# Autodesk Inventor assembly: cycloid_assy
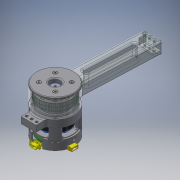
[picture p0: Inventor's stored thumbnail of the model, 180x180]
Saved by Autodesk Inventor 2019.4 (Build 234330000, 330)
## iProperties
Created: 2019-08-28
Part Number: cycloid_assy
Document SubType Name: Assembly
Designer: cdi
Author: cdi
## Documents named in this file (20)
- D:\SynologyDrive\workspace_inventor\2019_06_19.MT4008_actuator\[github_upload]\3d_print_cycloid_actuator_v2\inventor_file\cycloid_assy_v2.iam
- D:\SynologyDrive\workspace_inventor\2019_06_19.MT4008_actuator\[github_upload]\3d_print_cycloid_actuator_v2\inventor_file\bearing_18x12x4.ipt
- D:\SynologyDrive\workspace_inventor\2019_06_19.MT4008_actuator\[github_upload]\3d_print_cycloid_actuator_v2\inventor_file\cycloid_top_bottom_assy.iam
- D:\SynologyDrive\workspace_inventor\2019_06_19.MT4008_actuator\[github_upload]\3d_print_cycloid_actuator_v2\inventor_file\tarot-mt4008-motor-1.snapshot.3\inventor_export\Tarot 4008 Motor Assembly.iam
- D:\SynologyDrive\workspace_inventor\2019_06_19.MT4008_actuator\[github_upload]\3d_print_cycloid_actuator_v2\inventor_file\cycloid_housing.ipt
- D:\SynologyDrive\workspace_inventor\2019_06_19.MT4008_actuator\[github_upload]\3d_print_cycloid_actuator_v2\inventor_file\MJVESC_CIR_3D_Export\inv\MJVESC_MINI_VER03.ipt
- D:\SynologyDrive\workspace_inventor\2019_06_19.MT4008_actuator\[github_upload]\3d_print_cycloid_actuator_v2\inventor_file\AS5147_3D_Export\Inventor_AS5147_ENC_ANGLE_VER01\AS5147_ENC_ANGLE_VER01.iam
- D:\SynologyDrive\workspace_inventor\2019_06_19.MT4008_actuator\[github_upload]\3d_print_cycloid_actuator_v2\inventor_file\pin_3_22.ipt
- D:\SynologyDrive\workspace_inventor\2019_06_19.MT4008_actuator\[github_upload]\3d_print_cycloid_actuator_v2\inventor_file\bearing_52_40_7.ipt
- D:\SynologyDrive\workspace_inventor\2019_06_19.MT4008_actuator\[github_upload]\3d_print_cycloid_actuator_v2\inventor_file\cycloid_input_cam_onepart.ipt
- D:\SynologyDrive\workspace_inventor\2019_06_19.MT4008_actuator\[github_upload]\3d_print_cycloid_actuator_v2\inventor_file\cycloid_outter_motor_side.ipt
- D:\SynologyDrive\workspace_inventor\2019_06_19.MT4008_actuator\[github_upload]\3d_print_cycloid_actuator_v2\inventor_file\cycloid_outter_motor_opposite_side.ipt
- D:\SynologyDrive\workspace_inventor\2019_06_19.MT4008_actuator\[github_upload]\3d_print_cycloid_actuator_v2\inventor_file\cycloid_input_cam_motor_adapter.ipt
- D:\SynologyDrive\workspace_inventor\2019_06_19.MT4008_actuator\[github_upload]\3d_print_cycloid_actuator_v2\inventor_file\cycloid_outter_motor_fixer.ipt
- D:\SynologyDrive\workspace_inventor\2019_06_19.MT4008_actuator\[github_upload]\3d_print_cycloid_actuator_v2\inventor_file\magnet_6_2.5.ipt
- D:\SynologyDrive\workspace_inventor\2019_06_19.MT4008_actuator\[github_upload]\3d_print_cycloid_actuator_v2\inventor_file\cycloid_motor_controller_cover.ipt
- C:\Users\cdi\Documents\Inventor\Content Center Files\R2019\en-US\ASME ANSI B18.3.5M(2)\ASME_ANSI B18.3.5M - M3x30(2).ipt
- D:\SynologyDrive\workspace_inventor\2019_06_19.MT4008_actuator\[github_upload]\3d_print_cycloid_actuator_v2\inventor_file\motor_and_magnet_holder_new.ipt
- C:\Users\cdi\Documents\Inventor\Content Center Files\R2019\en-US\ASME ANSI B18.3.5M(2)\ASME_ANSI B18.3.5M - M3x8(2).ipt
- D:\SynologyDrive\workspace_inventor\2019_06_19.MT4008_actuator\[github_upload]\3d_print_cycloid_actuator_v2\inventor_file\as5047_holder_adder_5mm.ipt
## Components (27 placed, 19 different names)
1. AS5147_ENC_ANGLE_VER01:1 [sub-assembly] — Mate:188
2. as5047_holder_adder_5mm:1 — Mate:186, Mate:187, Mate:188, Mate:189
3. cycloid_input_cam_onepart:1 — Mate:118, Mate:124, Mate:125, Mate:126, Mate:127, Mate:161, Mate:163, Mate:164, Mate:165, Mate:177
4. Tarot 4008 Motor Assembly:1 [sub-assembly] — Mate:118, Mate:128, Mate:132, Mate:182, Mate:183
5. bearing_18x12x4:1 — Mate:157, Mate:158, Mate:161, Mate:163
6. cycloid_input_cam_motor_adapter:1 — Mate:124, Mate:125, Mate:126, Mate:127, Mate:128
7. cycloid_outter_motor_fixer:1 — Mate:132, Mate:141, Mate:175, Mate:176, Mate:178, Mate:184, Mate:185, Mate:186, Mate:187, Mate:189
8. magnet_6_2.5:2 — Mate:180, Flush:2
9. MJVESC_MINI_VER03:1 — Mate:138, Mate:141, Mate:178
10. bearing_52_40_7:3 — Mate:143, Mate:144, Mate:173
11. cycloid_top_bottom_assy:8 [sub-assembly] — Mate:160, Mate:177, Tangent:1, Tangent:3, Tangent:4, Tangent:5
12. cycloid_top_bottom_assy:10 [sub-assembly] — Mate:164, Mate:165, Tangent:2, Tangent:6, Tangent:7, Tangent:8
13. cycloid_outter_motor_opposite_side:1 — Mate:143, Mate:144, Mate:145, Mate:146, Mate:147, Mate:148, Mate:149, Mate:150, Mate:151, Mate:152, Mate:153, Mate:154, Mate:155, Mate:156, Mate:157, Mate:158, Mate:159, Mate:160, Mate:166
14. Broached Hexagon Socket Flat Countersunk Head Cap Screws - Metric M3x30:1 — Mate:145
15. Broached Hexagon Socket Flat Countersunk Head Cap Screws - Metric M3x30:2 — Mate:146
16. Broached Hexagon Socket Flat Countersunk Head Cap Screws - Metric M3x30:3 — Mate:147
17. Broached Hexagon Socket Flat Countersunk Head Cap Screws - Metric M3x30:4 — Mate:148
18. pin_3_22:7 — Mate:149, Mate:153, Mate:167, Mate:168, Tangent:1, Tangent:6
19. pin_3_22:8 — Mate:151, Mate:156, Tangent:2, Tangent:4
20. pin_3_22:9 — Mate:152, Mate:155, Tangent:5, Tangent:8
21. pin_3_22:10 — Mate:150, Mate:154, Tangent:3, Tangent:7
22. cycloid_housing:1 — Mate:116, Mate:172, Mate:173, Flush:1
23. cycloid_outter_motor_side:3 — Mate:166, Mate:167, Mate:168, Mate:169, Mate:170, Mate:184, Mate:185
24. bearing_52_40_7:4 — Mate:169, Mate:170, Mate:172, Flush:1
25. cycloid_motor_controller_cover:1 — Mate:175, Mate:176
26. motor_and_magnet_holder_new:1 — Mate:179, Mate:180, Mate:183, Flush:2
27. Broached Hexagon Socket Flat Countersunk Head Cap Screws - Metric M3x8:1 — Mate:179, Mate:182
## Relationships (63: Mate 53, Tangent 8, Flush 2)
- Mate:116: cycloid_housing:1
- Mate:118: cycloid_input_cam_onepart:1 ↔ Tarot 4008 Motor Assembly:1
- Mate:124: cycloid_input_cam_onepart:1 ↔ cycloid_input_cam_motor_adapter:1
- Mate:125: cycloid_input_cam_onepart:1 ↔ cycloid_input_cam_motor_adapter:1
- Mate:126: cycloid_input_cam_onepart:1 ↔ cycloid_input_cam_motor_adapter:1
- Mate:127: cycloid_input_cam_onepart:1 ↔ cycloid_input_cam_motor_adapter:1
- Mate:128: Tarot 4008 Motor Assembly:1 ↔ cycloid_input_cam_motor_adapter:1
- Mate:132: Tarot 4008 Motor Assembly:1 ↔ cycloid_outter_motor_fixer:1
- Mate:138: MJVESC_MINI_VER03:1
- Mate:141: cycloid_outter_motor_fixer:1 ↔ MJVESC_MINI_VER03:1
- Mate:143: bearing_52_40_7:3 ↔ cycloid_outter_motor_opposite_side:1
- Mate:144: bearing_52_40_7:3 ↔ cycloid_outter_motor_opposite_side:1
- Mate:145: cycloid_outter_motor_opposite_side:1 ↔ Broached Hexagon Socket Flat Countersunk Head Cap Screws - Metric M3x30:1
- Mate:146: cycloid_outter_motor_opposite_side:1 ↔ Broached Hexagon Socket Flat Countersunk Head Cap Screws - Metric M3x30:2
- Mate:147: cycloid_outter_motor_opposite_side:1 ↔ Broached Hexagon Socket Flat Countersunk Head Cap Screws - Metric M3x30:3
- Mate:148: cycloid_outter_motor_opposite_side:1 ↔ Broached Hexagon Socket Flat Countersunk Head Cap Screws - Metric M3x30:4
- Mate:149: cycloid_outter_motor_opposite_side:1 ↔ pin_3_22:7
- Mate:150: cycloid_outter_motor_opposite_side:1 ↔ pin_3_22:10
- Mate:151: cycloid_outter_motor_opposite_side:1 ↔ pin_3_22:8
- Mate:152: cycloid_outter_motor_opposite_side:1 ↔ pin_3_22:9
- Mate:153: cycloid_outter_motor_opposite_side:1 ↔ pin_3_22:7
- Mate:154: cycloid_outter_motor_opposite_side:1 ↔ pin_3_22:10
- Mate:155: cycloid_outter_motor_opposite_side:1 ↔ pin_3_22:9
- Mate:156: cycloid_outter_motor_opposite_side:1 ↔ pin_3_22:8
- Mate:157: bearing_18x12x4:1 ↔ cycloid_outter_motor_opposite_side:1
- Mate:158: bearing_18x12x4:1 ↔ cycloid_outter_motor_opposite_side:1
- Mate:159: cycloid_outter_motor_opposite_side:1
- Mate:160 (0.5 mm): cycloid_top_bottom_assy:8 ↔ cycloid_outter_motor_opposite_side:1
- Mate:161: cycloid_input_cam_onepart:1 ↔ bearing_18x12x4:1
- Mate:163: cycloid_input_cam_onepart:1 ↔ bearing_18x12x4:1
- Mate:164: cycloid_input_cam_onepart:1 ↔ cycloid_top_bottom_assy:10
- Mate:165: cycloid_input_cam_onepart:1 ↔ cycloid_top_bottom_assy:10
- Mate:166: cycloid_outter_motor_opposite_side:1 ↔ cycloid_outter_motor_side:3
- Mate:167: pin_3_22:7 ↔ cycloid_outter_motor_side:3
- Mate:168: pin_3_22:7 ↔ cycloid_outter_motor_side:3
- Mate:169: cycloid_outter_motor_side:3 ↔ bearing_52_40_7:4
- Mate:170: cycloid_outter_motor_side:3 ↔ bearing_52_40_7:4
- Mate:172: cycloid_housing:1 ↔ bearing_52_40_7:4
- Mate:173: bearing_52_40_7:3 ↔ cycloid_housing:1
- Flush:1: cycloid_housing:1 ↔ bearing_52_40_7:4
- Mate:175: cycloid_outter_motor_fixer:1 ↔ cycloid_motor_controller_cover:1
- Mate:176: cycloid_outter_motor_fixer:1 ↔ cycloid_motor_controller_cover:1
- Mate:177: cycloid_input_cam_onepart:1 ↔ cycloid_top_bottom_assy:8
- Tangent:1: cycloid_top_bottom_assy:8 ↔ pin_3_22:7
- Tangent:2: cycloid_top_bottom_assy:10 ↔ pin_3_22:8
- Tangent:3: cycloid_top_bottom_assy:8 ↔ pin_3_22:10
- Tangent:4: cycloid_top_bottom_assy:8 ↔ pin_3_22:8
- Tangent:5: cycloid_top_bottom_assy:8 ↔ pin_3_22:9
- Tangent:6: cycloid_top_bottom_assy:10 ↔ pin_3_22:7
- Tangent:7: cycloid_top_bottom_assy:10 ↔ pin_3_22:10
- Tangent:8: cycloid_top_bottom_assy:10 ↔ pin_3_22:9
- Mate:178: cycloid_outter_motor_fixer:1 ↔ MJVESC_MINI_VER03:1
- Mate:179: motor_and_magnet_holder_new:1 ↔ Broached Hexagon Socket Flat Countersunk Head Cap Screws - Metric M3x8:1
- Mate:180: magnet_6_2.5:2 ↔ motor_and_magnet_holder_new:1
- Mate:182: Tarot 4008 Motor Assembly:1 ↔ Broached Hexagon Socket Flat Countersunk Head Cap Screws - Metric M3x8:1
- Mate:183: Tarot 4008 Motor Assembly:1 ↔ motor_and_magnet_holder_new:1
- Flush:2: magnet_6_2.5:2 ↔ motor_and_magnet_holder_new:1
- Mate:184: cycloid_outter_motor_fixer:1 ↔ cycloid_outter_motor_side:3
- Mate:185: cycloid_outter_motor_fixer:1 ↔ cycloid_outter_motor_side:3
- Mate:186: as5047_holder_adder_5mm:1 ↔ cycloid_outter_motor_fixer:1
- Mate:187: as5047_holder_adder_5mm:1 ↔ cycloid_outter_motor_fixer:1
- Mate:188: AS5147_ENC_ANGLE_VER01:1 ↔ as5047_holder_adder_5mm:1
- Mate:189: as5047_holder_adder_5mm:1 ↔ cycloid_outter_motor_fixer:1
